# Autodesk Inventor assembly: OmniWheel
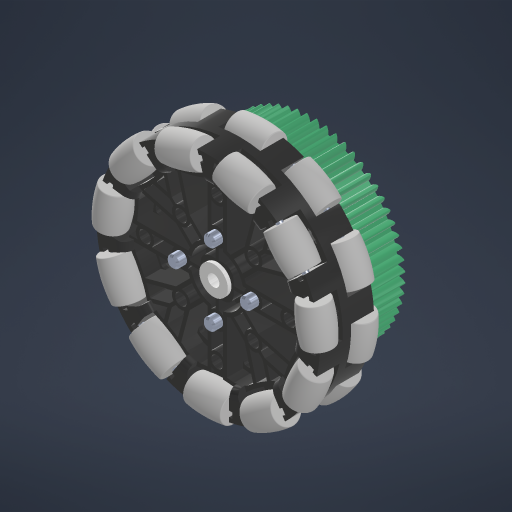
[picture p0: Inventor's stored thumbnail of the model, 512x512]
Saved by Autodesk Inventor 2023 (Build 270158000, 158)
## iProperties
Created: 2023-05-09
Part Number: OmniWheel
Document SubType Name: Assembly
Designer: alex
Author: alex
## Documents named in this file (8)
- C:\Users\alex\Documents\GitHub\4067X-Over-Under-CAD\Chassis\OmniWheel.iam
- C:\Users\alex\Documents\GitHub\4067X-Over-Under-CAD\VEX-CAD-Inventor\Motion\Gears\HS Gear\HS 60T Gear, Circle Old.ipt
- C:\Users\alex\Documents\GitHub\4067X-Over-Under-CAD\VEX-CAD-Inventor\Structure\Standoff\Standoff .50.ipt
- C:\Users\alex\Documents\GitHub\4067X-Over-Under-CAD\VEX-CAD-Inventor\Structure\Standoff.ipt
- C:\Users\alex\Documents\GitHub\4067X-Over-Under-CAD\VEX-CAD-Inventor\Motion\Wheels\Omni Wheel\3.25 Omni AS, Circle.iam
- C:\Users\alex\Documents\GitHub\4067X-Over-Under-CAD\VEX-CAD-Inventor\Motion\Wheels\Omni Wheel.iam
- C:\Users\alex\Documents\GitHub\4067X-Over-Under-CAD\VEX-CAD-Inventor\Structure\Hardware\Screw Steel - Star\SScrew Star Smooth 1.250.ipt
- C:\Users\alex\Documents\GitHub\4067X-Over-Under-CAD\VEX-CAD-Inventor\Structure\Hardware\Screw Steel - Star.ipt
## Components (10 placed, 4 different names)
1. HS 60T Gear, Circle Old:1 — Insert:1, Insert:2, Insert:3, Insert:4, Insert:7, Insert:8, Insert:9, Insert:10
2. Standoff .50:1 — Insert:1, Insert:6
3. Standoff .50:2 — Insert:2
4. Standoff .50:3 — Insert:3, Insert:5
5. Standoff .50:4 — Insert:4
6. 3.25 Omni AS, Circle:1 [sub-assembly] — Insert:5, Insert:6
7. SScrew Star Smooth 1.250:1 — Insert:7
8. SScrew Star Smooth 1.250:2 — Insert:8
9. SScrew Star Smooth 1.250:3 — Insert:9
10. SScrew Star Smooth 1.250:4 — Insert:10
## Relationships (10: Insert 10)
- Insert:1: HS 60T Gear, Circle Old:1 ↔ Standoff .50:1
- Insert:2: HS 60T Gear, Circle Old:1 ↔ Standoff .50:2
- Insert:3: HS 60T Gear, Circle Old:1 ↔ Standoff .50:3
- Insert:4: HS 60T Gear, Circle Old:1 ↔ Standoff .50:4
- Insert:5: Standoff .50:3 ↔ 3.25 Omni AS, Circle:1
- Insert:6: Standoff .50:1 ↔ 3.25 Omni AS, Circle:1
- Insert:7: HS 60T Gear, Circle Old:1 ↔ SScrew Star Smooth 1.250:1
- Insert:8: HS 60T Gear, Circle Old:1 ↔ SScrew Star Smooth 1.250:2
- Insert:9: HS 60T Gear, Circle Old:1 ↔ SScrew Star Smooth 1.250:3
- Insert:10: HS 60T Gear, Circle Old:1 ↔ SScrew Star Smooth 1.250:4
